# Autodesk Inventor assembly: Banhxenew
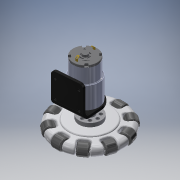
[picture p0: Inventor's stored thumbnail of the model, 180x180]
Saved by Autodesk Inventor 2019 (Build 230136000, 136)
## iProperties
Created: 2021-01-20
Part Number: Banhxenew
Document SubType Name: Assembly
Designer: Admin
Author: Admin
## Documents named in this file (5)
- C:\Users\Admin\Documents\Inventor\Doan\Banhxenew.iam
- C:\Users\Admin\Documents\Inventor\Doan\Hubnew.ipt
- C:\Users\Admin\Documents\Inventor\Doan\Omninew.ipt
- C:\Users\Admin\Documents\Inventor\Doan\JGB37-520.iam
- C:\Users\Admin\Documents\Inventor\Doan\JGB37-520 12 v metal geared motor bracket.ipt
## Components (4 placed, 4 different names)
1. Hubnew:1 — Mate:1, Mate:2, Mate:3, Mate:7, Mate:8, Mate:9, Mate:10
2. Omninew:1 — Mate:1, Mate:2, Mate:3
3. JGB37-520:1 [sub-assembly] — Mate:4, Mate:5, Mate:6, Mate:7, Mate:8, Mate:9, Mate:10
4. JGB37-520 12 v metal geared motor bracket:1 — Mate:4, Mate:5, Mate:6
## Relationships (10: Mate 10)
- Mate:1: Hubnew:1 ↔ Omninew:1
- Mate:2: Hubnew:1 ↔ Omninew:1
- Mate:3: Hubnew:1 ↔ Omninew:1
- Mate:4: JGB37-520:1 ↔ JGB37-520 12 v metal geared motor bracket:1
- Mate:5: JGB37-520:1 ↔ JGB37-520 12 v metal geared motor bracket:1
- Mate:6: JGB37-520:1 ↔ JGB37-520 12 v metal geared motor bracket:1
- Mate:7: Hubnew:1 ↔ JGB37-520:1
- Mate:8: Hubnew:1 ↔ JGB37-520:1
- Mate:9: Hubnew:1 ↔ JGB37-520:1
- Mate:10: Hubnew:1 ↔ JGB37-520:1
